# Autodesk Inventor assembly: 090 ASY bottom
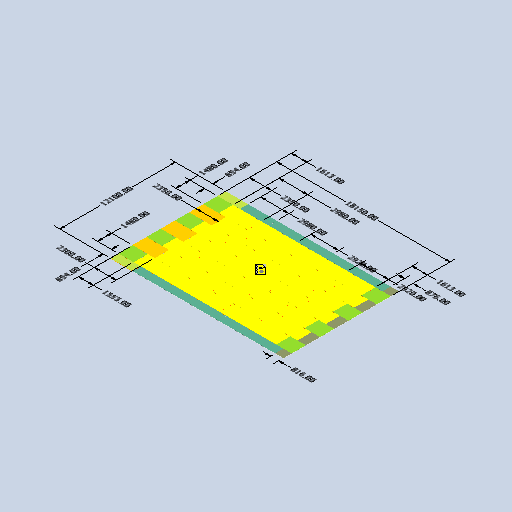
[picture p0: Inventor's stored thumbnail of the model, 512x512]
Saved by Autodesk Inventor 2026 (Build 300175000, 175)
## iProperties
Created: 2026-05-19
Part Number: 090 ASY bottom
Document SubType Name: Assembly
Designer: user
Mass: 1.0309e+07 g
Surface Area: 5.30613e+06 cm^2
Volume: 1.31325e+06 cm^3
Density: 7.85 g/cm^3
Author: user
## Documents named in this file (12)
- C:\Users\user\Documents\Inventor\GBK-Gubkinskiy\090 ASY bottom.iam
- C:\Users\user\Documents\Inventor\GBK-Gubkinskiy\Пол\GBK bottom 0124.ipt
- C:\Users\user\Documents\Inventor\GBK-Gubkinskiy\Пол\GBK bottom 0125.ipt
- C:\Users\user\Documents\Inventor\GBK-Gubkinskiy\Пол\GBK bottom 0112.ipt
- C:\Users\user\Documents\Inventor\GBK-Gubkinskiy\Пол\GBK bottom 0127.ipt
- C:\Users\user\Documents\Inventor\GBK-Gubkinskiy\ASY GBK bottom 0010.iam
- C:\Users\user\Documents\Inventor\GBK-Gubkinskiy\ASY GBK bottom 0020.iam
- C:\Users\user\Documents\Inventor\GBK-Gubkinskiy\ASY GBK bottom 0021.iam
- C:\Users\user\Documents\Inventor\GBK-Gubkinskiy\ASY GBK bottom 0022.iam
- C:\Users\user\Documents\Inventor\GBK-Gubkinskiy\ASY GBK bottom 0023.iam
- C:\Users\user\Documents\Inventor\GBK-Gubkinskiy\ASY GBK bottom 0021_CPY.iam
- C:\Users\user\Documents\Inventor\GBK-Gubkinskiy\ASY GBK bottom 0024.iam
## Components (71 placed, 11 different names)
1. GBK bottom 0123:5
2. GBK bottom 0127:1 — Жесткий:22
3. GBK bottom 0124:2 — Жесткий:7
4. GBK bottom 0125:10 — Жесткий:22
5. GBK bottom 0125:5 — Жесткий:6, Жесткий:7
6. GBK bottom 0125:9
7. GBK bottom 0125:4 — Жесткий:6
8. GBK bottom 0125:8
9. ASY GBK bottom 0010:3 [sub-assembly] — Жесткий:54
10. ASY GBK bottom 0010:2 [sub-assembly] — Жесткий:37, Жесткий:50
11. ASY GBK bottom 0010:1 [sub-assembly] — Жесткий:37
12. ASY GBK bottom 0020:1 [sub-assembly] — Жесткий:45
13. ASY GBK bottom 0020:2 [sub-assembly] — Жесткий:45, Жесткий:46
14. ASY GBK bottom 0020:3 [sub-assembly] — Жесткий:46, Жесткий:48
15. ASY GBK bottom 0020:4 [sub-assembly] — Жесткий:48, Жесткий:49
16. ASY GBK bottom 0020:5 [sub-assembly] — Жесткий:49, Жесткий:94
17. ASY GBK bottom 0021:1 [sub-assembly] — Жесткий:94
18. ASY GBK bottom 0022:1 [sub-assembly]
19. ASY GBK bottom 0023:1 [sub-assembly]
20. ASY GBK bottom 0010:4 [sub-assembly] — Жесткий:50, Жесткий:51
21. ASY GBK bottom 0010:5 [sub-assembly] — Жесткий:51, Жесткий:52
22. ASY GBK bottom 0010:6 [sub-assembly] — Жесткий:52, Жесткий:53
23. ASY GBK bottom 0023:2 [sub-assembly] — Жесткий:53
24. ASY GBK bottom 0010:7 [sub-assembly] — Жесткий:54, Жесткий:55
25. ASY GBK bottom 0010:8 [sub-assembly] — Жесткий:55, Жесткий:56
26. ASY GBK bottom 0010:9 [sub-assembly] — Жесткий:56, Жесткий:57
27. ASY GBK bottom 0010:10 [sub-assembly] — Жесткий:57, Жесткий:58
28. ASY GBK bottom 0025:1 [sub-assembly] — Жесткий:58
29. ASY GBK bottom 0010:11 [sub-assembly]
30. ASY GBK bottom 0010:12 [sub-assembly]
31. ASY GBK bottom 0023:3 [sub-assembly] — Жесткий:72
32. ASY GBK bottom 0010:13 [sub-assembly]
33. ASY GBK bottom 0010:14 [sub-assembly]
34. ASY GBK bottom 0010:15 [sub-assembly]
35. ASY GBK bottom 0023:4 [sub-assembly]
36. ASY GBK bottom 0024:1 [sub-assembly]
37. ASY GBK bottom 0010:16 [sub-assembly]
38. ASY GBK bottom 0010:17 [sub-assembly]
39. ASY GBK bottom 0010:18 [sub-assembly]
40. ASY GBK bottom 0010:19 [sub-assembly]
41. ASY GBK bottom 0010:20 [sub-assembly]
42. ASY GBK bottom 0025:2 [sub-assembly]
43. ASY GBK bottom 0024:2 [sub-assembly] — Жесткий:72, Жесткий:79
44. ASY GBK bottom 0010:21 [sub-assembly]
45. ASY GBK bottom 0010:22 [sub-assembly]
46. ASY GBK bottom 0023:5 [sub-assembly] — Жесткий:79, Жесткий:86
47. ASY GBK bottom 0010:23 [sub-assembly]
48. ASY GBK bottom 0010:24 [sub-assembly]
49. ASY GBK bottom 0010:25 [sub-assembly]
50. ASY GBK bottom 0023:6 [sub-assembly]
51. ASY GBK bottom 0010:26 [sub-assembly]
52. ASY GBK bottom 0010:27 [sub-assembly]
53. ASY GBK bottom 0010:28 [sub-assembly]
54. ASY GBK bottom 0010:29 [sub-assembly]
55. ASY GBK bottom 0010:30 [sub-assembly]
56. ASY GBK bottom 0025:3 [sub-assembly]
57. ASY GBK bottom 0024:3 [sub-assembly] — Жесткий:86, Жесткий:93
58. ASY GBK bottom 0010:31 [sub-assembly]
59. ASY GBK bottom 0010:32 [sub-assembly]
60. ASY GBK bottom 0023:7 [sub-assembly] — Жесткий:93, Жесткий:101
61. ASY GBK bottom 0010:33 [sub-assembly]
62. ASY GBK bottom 0010:34 [sub-assembly]
63. ASY GBK bottom 0010:35 [sub-assembly]
64. ASY GBK bottom 0023:8 [sub-assembly]
65. ASY GBK bottom 0020:6 [sub-assembly]
66. ASY GBK bottom 0020:7 [sub-assembly]
67. ASY GBK bottom 0020:8 [sub-assembly]
68. ASY GBK bottom 0020:9 [sub-assembly]
69. ASY GBK bottom 0020:10 [sub-assembly]
70. ASY GBK bottom 0021:2 [sub-assembly]
71. ASY GBK bottom 0022:2 [sub-assembly] — Жесткий:101
## Relationships (71: WeldJoint 68, Mate 3)
- [WeldJoint] (4 mm): ASY GBK bottom 0010:1 ↔ ASY GBK bottom 0023:1
- Жесткий:6 [WeldJoint] (4 mm): GBK bottom 0125:5 ↔ GBK bottom 0125:4
- Жесткий:7 [WeldJoint] (4 mm): GBK bottom 0124:2 ↔ GBK bottom 0125:5
- [Mate] (-9075 mm): ASY GBK bottom 0023:1
- [WeldJoint] (4 mm): GBK bottom 0125:9 ↔ GBK bottom 0125:8
- [WeldJoint] (4 mm): GBK bottom 0125:10 ↔ GBK bottom 0125:9
- [WeldJoint] (4 mm): ASY GBK bottom 0022:1 ↔ ASY GBK bottom 0023:1
- [Mate]: ASY GBK bottom 0022:1
- [Mate] (-6050 mm): ASY GBK bottom 0022:1
- [WeldJoint] (4 mm): ASY GBK bottom 0020:1 ↔ ASY GBK bottom 0022:1
- [WeldJoint] (4 mm): ASY GBK bottom 0023:1 ↔ ASY GBK bottom 0024:1
- [WeldJoint] (4 mm): GBK bottom 0123:5 ↔ ASY GBK bottom 0021:1
- Жесткий:22 [WeldJoint] (4 mm): GBK bottom 0127:1 ↔ GBK bottom 0125:10
- Жесткий:37 [WeldJoint] (4 mm): ASY GBK bottom 0010:2 ↔ ASY GBK bottom 0010:1
- [WeldJoint] (4 mm): ASY GBK bottom 0010:3 ↔ ASY GBK bottom 0024:1
- Жесткий:45 [WeldJoint] (4 mm): ASY GBK bottom 0020:1 ↔ ASY GBK bottom 0020:2
- Жесткий:46 [WeldJoint] (4 mm): ASY GBK bottom 0020:2 ↔ ASY GBK bottom 0020:3
- Жесткий:48 [WeldJoint] (4 mm): ASY GBK bottom 0020:3 ↔ ASY GBK bottom 0020:4
- Жесткий:49 [WeldJoint] (4 mm): ASY GBK bottom 0020:4 ↔ ASY GBK bottom 0020:5
- Жесткий:50 [WeldJoint] (4 mm): ASY GBK bottom 0010:2 ↔ ASY GBK bottom 0010:4
- Жесткий:51 [WeldJoint] (4 mm): ASY GBK bottom 0010:4 ↔ ASY GBK bottom 0010:5
- Жесткий:52 [WeldJoint] (4 mm): ASY GBK bottom 0010:5 ↔ ASY GBK bottom 0010:6
- Жесткий:53 [WeldJoint] (4 mm): ASY GBK bottom 0010:6 ↔ ASY GBK bottom 0023:2
- Жесткий:54 [WeldJoint] (4 mm): ASY GBK bottom 0010:3 ↔ ASY GBK bottom 0010:7
- Жесткий:55 [WeldJoint] (4 mm): ASY GBK bottom 0010:7 ↔ ASY GBK bottom 0010:8
- Жесткий:56 [WeldJoint] (4 mm): ASY GBK bottom 0010:8 ↔ ASY GBK bottom 0010:9
- Жесткий:57 [WeldJoint] (4 mm): ASY GBK bottom 0010:9 ↔ ASY GBK bottom 0010:10
- Жесткий:58 [WeldJoint] (4 mm): ASY GBK bottom 0010:10 ↔ ASY GBK bottom 0025:1
- [WeldJoint] (4 mm): ASY GBK bottom 0010:11 ↔ ASY GBK bottom 0023:3
- [WeldJoint] (4 mm): ASY GBK bottom 0010:11 ↔ ASY GBK bottom 0010:12
- [WeldJoint] (4 mm): ASY GBK bottom 0010:12 ↔ ASY GBK bottom 0010:13
- [WeldJoint] (4 mm): ASY GBK bottom 0010:13 ↔ ASY GBK bottom 0010:14
- [WeldJoint] (4 mm): ASY GBK bottom 0010:14 ↔ ASY GBK bottom 0010:15
- [WeldJoint] (4 mm): ASY GBK bottom 0010:15 ↔ ASY GBK bottom 0023:4
- [WeldJoint] (4 mm): ASY GBK bottom 0023:3 ↔ ASY GBK bottom 0024:1
- [WeldJoint] (4 mm): ASY GBK bottom 0010:16 ↔ ASY GBK bottom 0024:2
- [WeldJoint] (4 mm): ASY GBK bottom 0010:16 ↔ ASY GBK bottom 0010:17
- [WeldJoint] (4 mm): ASY GBK bottom 0010:17 ↔ ASY GBK bottom 0010:18
- [WeldJoint] (4 mm): ASY GBK bottom 0010:18 ↔ ASY GBK bottom 0010:19
- [WeldJoint] (4 mm): ASY GBK bottom 0010:19 ↔ ASY GBK bottom 0010:20
- [WeldJoint] (4 mm): ASY GBK bottom 0010:20 ↔ ASY GBK bottom 0025:2
- Жесткий:72 [WeldJoint] (4 mm): ASY GBK bottom 0023:3 ↔ ASY GBK bottom 0024:2
- [WeldJoint] (4 mm): ASY GBK bottom 0010:21 ↔ ASY GBK bottom 0023:5
- [WeldJoint] (4 mm): ASY GBK bottom 0010:21 ↔ ASY GBK bottom 0010:22
- [WeldJoint] (4 mm): ASY GBK bottom 0010:22 ↔ ASY GBK bottom 0010:23
- [WeldJoint] (4 mm): ASY GBK bottom 0010:23 ↔ ASY GBK bottom 0010:24
- [WeldJoint] (4 mm): ASY GBK bottom 0010:24 ↔ ASY GBK bottom 0010:25
- [WeldJoint] (4 mm): ASY GBK bottom 0010:25 ↔ ASY GBK bottom 0023:6
- Жесткий:79 [WeldJoint] (4 mm): ASY GBK bottom 0024:2 ↔ ASY GBK bottom 0023:5
- [WeldJoint] (4 mm): ASY GBK bottom 0010:26 ↔ ASY GBK bottom 0024:3
- [WeldJoint] (4 mm): ASY GBK bottom 0010:26 ↔ ASY GBK bottom 0010:27
- [WeldJoint] (4 mm): ASY GBK bottom 0010:27 ↔ ASY GBK bottom 0010:28
- [WeldJoint] (4 mm): ASY GBK bottom 0010:28 ↔ ASY GBK bottom 0010:29
- [WeldJoint] (4 mm): ASY GBK bottom 0010:29 ↔ ASY GBK bottom 0010:30
- [WeldJoint] (4 mm): ASY GBK bottom 0010:30 ↔ ASY GBK bottom 0025:3
- Жесткий:86 [WeldJoint] (4 mm): ASY GBK bottom 0023:5 ↔ ASY GBK bottom 0024:3
- [WeldJoint] (4 mm): ASY GBK bottom 0010:31 ↔ ASY GBK bottom 0023:7
- [WeldJoint] (4 mm): ASY GBK bottom 0010:31 ↔ ASY GBK bottom 0010:32
- [WeldJoint] (4 mm): ASY GBK bottom 0010:32 ↔ ASY GBK bottom 0010:33
- [WeldJoint] (4 mm): ASY GBK bottom 0010:33 ↔ ASY GBK bottom 0010:34
- [WeldJoint] (4 mm): ASY GBK bottom 0010:34 ↔ ASY GBK bottom 0010:35
- [WeldJoint] (4 mm): ASY GBK bottom 0010:35 ↔ ASY GBK bottom 0023:8
- Жесткий:93 [WeldJoint] (4 mm): ASY GBK bottom 0024:3 ↔ ASY GBK bottom 0023:7
- Жесткий:94 [WeldJoint] (4 mm): ASY GBK bottom 0020:5 ↔ ASY GBK bottom 0021:1
- [WeldJoint] (4 mm): ASY GBK bottom 0020:6 ↔ ASY GBK bottom 0022:2
- [WeldJoint] (4 mm): ASY GBK bottom 0020:6 ↔ ASY GBK bottom 0020:7
- [WeldJoint] (4 mm): ASY GBK bottom 0020:7 ↔ ASY GBK bottom 0020:8
- [WeldJoint] (4 mm): ASY GBK bottom 0020:8 ↔ ASY GBK bottom 0020:9
- [WeldJoint] (4 mm): ASY GBK bottom 0020:9 ↔ ASY GBK bottom 0020:10
- [WeldJoint] (4 mm): ASY GBK bottom 0020:10 ↔ ASY GBK bottom 0021:2
- Жесткий:101 [WeldJoint] (4 mm): ASY GBK bottom 0023:7 ↔ ASY GBK bottom 0022:2
## Named parameters: d66_d60 = 4 mm, d67_d61 = 4 mm, d154_d147 = 4 mm, d155_d148 = 4 mm, d156_d111 = 4 mm, d157_d145 = 4 mm, d158_d146 = 4 mm, d159_d37 = 4 mm, d161_d149 = 4 mm, d162_d150 = 4 mm, d163_d151 = 4 mm, d164_d152 = 4 mm, d165_d153 = 4 mm, d166_d113 = 4 mm, d168_d147 = 4 mm, d169_d148 = 4 mm, d170_d111 = 4 mm, d171_d145 = 4 mm, d172_d146 = 4 mm, d173_d37 = 4 mm, d175_d149 = 4 mm, d176_d150 = 4 mm, d177_d151 = 4 mm, d178_d152 = 4 mm, d179_d153 = 4 mm, d180_d113 = 4 mm, d188_d147 = 4 mm, d189_d148 = 4 mm, d190_d111 = 4 mm, d191_d145 = 4 mm, d192_d146 = 4 mm, d193_d37 = 4 mm, d196_d195 = 4 mm, d197_d137 = 4 mm, d198_d138 = 4 mm, d199_d140 = 4 mm, d200_d141 = 4 mm, d201_d76 = 4 mm
